# Autodesk Inventor assembly: CheckValve+Reg 1.0
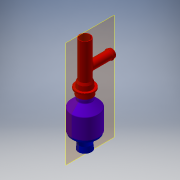
[picture p0: Inventor's stored thumbnail of the model, 180x180]
Saved by Autodesk Inventor 2019 (Build 230136000, 136)
## iProperties
Created: 2019-04-04
Part Number: CheckValve+Reg 1.0
Document SubType Name: Assembly
Designer: Kepler
Author: Kepler
## Documents named in this file (5)
- C:\Users\Kepler\Documents\Inventor\Whistles\CheckValve+Reg 1.0.iam
- C:\Users\Kepler\Documents\Inventor\Whistles\CheckBallonWindbox Connecter 1.0.ipt
- C:\Users\Kepler\Documents\Inventor\Whistles\CheckValve 1.0.ipt
- C:\Users\Kepler\Documents\Inventor\Whistles\CheckValveValve1.0.ipt
- C:\Users\Kepler\Documents\Inventor\Whistles\CheckValve Endcap 1.0.ipt
## Components (4 placed, 4 different names)
1. CheckBallonWindbox Connecter 1.0:1 — Mate:1, Mate:2, Rotation:1
2. CheckValve 1.0:1 — Mate:1, Mate:2, Mate:3, Mate:4, Mate:5, Mate:6, Rotation:1
3. CheckValveValve1.0:1 — Mate:3, Mate:4
4. CheckValve Endcap 1.0:1 — Mate:5, Mate:6
## Relationships (8: Mate 6, Flush 1, RelateRotation 1)
- Mate:1: CheckBallonWindbox Connecter 1.0:1 ↔ CheckValve 1.0:1
- Mate:2 (1 mm): CheckBallonWindbox Connecter 1.0:1 ↔ CheckValve 1.0:1
- Mate:3: CheckValve 1.0:1 ↔ CheckValveValve1.0:1
- Mate:4: CheckValve 1.0:1 ↔ CheckValveValve1.0:1
- Mate:5: CheckValve 1.0:1 ↔ CheckValve Endcap 1.0:1
- Mate:6: CheckValve 1.0:1 ↔ CheckValve Endcap 1.0:1
- Flush:1 (-3 mm)
- Rotation:1 [RelateRotation] (1 ul): CheckBallonWindbox Connecter 1.0:1 ↔ CheckValve 1.0:1
